# Autodesk Inventor assembly: Beefer_Montiert
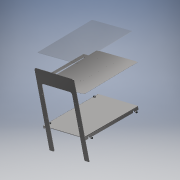
[picture p0: Inventor's stored thumbnail of the model, 180x180]
Saved by Autodesk Inventor 2018 (Build 220112000, 112)
## iProperties
Created: 2017-10-08
Part Number: Beefer_Montiert
Material: Generisch
Document SubType Name: Assembly
Designer: jro
Mass: 245.166 g
Surface Area: 2512.49 cm^2
Volume: 245.166 cm^3
Density: 1 g/cm^3
Author: jro
## Documents named in this file (13)
- C:\OneDrive\Beefer\Beefer_Montiert.iam
- C:\OneDrive\Beefer\Boden.ipt
- C:\OneDrive\Beefer\Front.ipt
- C:\OneDrive\Beefer\SeiteLinks.ipt
- C:\OneDrive\Beefer\SeiteRechts.ipt
- C:\OneDrive\Beefer\RueckWand.ipt
- C:\OneDrive\Beefer\Deckel.ipt
- C:\OneDrive\Beefer\BrennerHalter.ipt
- C:\OneDrive\Beefer\Gegenhalter.ipt
- C:\OneDrive\Beefer\EinschubRechts.ipt
- C:\OneDrive\Beefer\MutterMitUScheibe.ipt
- C:\Users\kuckal\Documents\Inventor\Content Center Files\R2018\de-DE\ISO 7380-1\ISO 7380-1 - M4 x 6.ipt
- C:\OneDrive\Beefer\BodenV2.ipt
## Components (18 placed, 12 different names)
1. Boden:1 — Fluchtend:1, Fluchtend:2, Fluchtend:3, Fluchtend:13, Fluchtend:14, Fluchtend:15, Fluchtend:16
2. Front:2 — Fluchtend:13, Fluchtend:14, Passend:11
3. SeiteLinks:1 — Fluchtend:8, Fluchtend:9, Passend:6, Passend:7, Passend:8, Passend:9, Einfügen:3, Einfügen:4
4. SeiteRechts:1 — Fluchtend:10, Fluchtend:11, Passend:2, Passend:3, Passend:4, Passend:5, Einfügen:1, Einfügen:2, Fluchtend:17
5. RueckWand:1 — Fluchtend:8, Fluchtend:9
6. Deckel:1 — Fluchtend:10, Fluchtend:11
7. BrennerHalter:1 — Passend:10
8. Gegenhalter:1 — Passend:10, Passend:11
9. EinschubRechts:1 — Fluchtend:15, Fluchtend:16
10. MutterMitUScheibe:1 — Passend:3, Passend:5
11. MutterMitUScheibe:2 — Passend:2, Passend:4
12. ISO 7380-1 M4 x 6:1 — Einfügen:1
13. ISO 7380-1 M4 x 6:2 — Einfügen:2
14. MutterMitUScheibe:3 — Passend:7, Passend:8
15. MutterMitUScheibe:4 — Passend:6, Passend:9
16. ISO 7380-1 M4 x 6:3 — Einfügen:3
17. ISO 7380-1 M4 x 6:4 — Einfügen:4
18. BodenV2:1 — Fluchtend:18, Fluchtend:19
## Relationships (32: Flush 18, Mate 10, Insert 4)
- Fluchtend:1 [Flush]: Boden:1
- Fluchtend:2 [Flush]: Boden:1
- Fluchtend:3 [Flush]: Boden:1
- [Flush] (-124 mm): Front:2
- [Flush] (3.037 mm): Front:2 ↔ SeiteLinks:1
- [Flush]: Front:2 ↔ SeiteRechts:1
- Fluchtend:8 [Flush]: SeiteLinks:1 ↔ RueckWand:1
- Fluchtend:9 [Flush]: SeiteLinks:1 ↔ RueckWand:1
- Fluchtend:10 [Flush]: SeiteRechts:1 ↔ Deckel:1
- Fluchtend:11 [Flush]: SeiteRechts:1 ↔ Deckel:1
- [Flush] (-5 mm): Front:2 ↔ BrennerHalter:1
- Fluchtend:13 [Flush] (5 mm): Boden:1 ↔ Front:2
- Fluchtend:14 [Flush] (5 mm): Boden:1 ↔ Front:2
- Fluchtend:15 [Flush]: Boden:1 ↔ EinschubRechts:1
- Fluchtend:16 [Flush]: Boden:1 ↔ EinschubRechts:1
- Passend:2 [Mate]: SeiteRechts:1 ↔ MutterMitUScheibe:2
- Passend:3 [Mate]: SeiteRechts:1 ↔ MutterMitUScheibe:1
- Passend:4 [Mate]: SeiteRechts:1 ↔ MutterMitUScheibe:2
- Passend:5 [Mate]: SeiteRechts:1 ↔ MutterMitUScheibe:1
- Einfügen:1 [Insert]: SeiteRechts:1 ↔ ISO 7380-1 M4 x 6:1
- Einfügen:2 [Insert]: SeiteRechts:1 ↔ ISO 7380-1 M4 x 6:2
- Passend:6 [Mate]: SeiteLinks:1 ↔ MutterMitUScheibe:4
- Passend:7 [Mate]: SeiteLinks:1 ↔ MutterMitUScheibe:3
- Passend:8 [Mate]: SeiteLinks:1 ↔ MutterMitUScheibe:3
- Passend:9 [Mate]: SeiteLinks:1 ↔ MutterMitUScheibe:4
- Einfügen:3 [Insert]: SeiteLinks:1 ↔ ISO 7380-1 M4 x 6:3
- Einfügen:4 [Insert]: SeiteLinks:1 ↔ ISO 7380-1 M4 x 6:4
- Fluchtend:17 [Flush] (-25 mm): SeiteRechts:1
- Fluchtend:18 [Flush]: BodenV2:1
- Fluchtend:19 [Flush]: BodenV2:1
- Passend:10 [Mate]: BrennerHalter:1 ↔ Gegenhalter:1
- Passend:11 [Mate] (28.5 mm): Front:2 ↔ Gegenhalter:1
## Named parameters: FrontPortalAbstand = -124 mm
